# Autodesk Inventor assembly: Overall_Assembly_Rev2
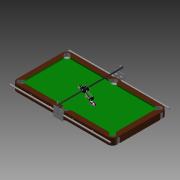
[picture p0: Inventor's stored thumbnail of the model, 180x180]
Saved by Autodesk Inventor 2015 (Build 190159000, 159)
## iProperties
Created: 2016-12-23
Part Number: Overall_Assembly_Rev2
Document SubType Name: Assembly
Designer: Guy
Author: Guy
## Documents named in this file (6)
- C:\Users\Ernest\Documents\Capstone-Project\doc\CAD\LowLevel_Rev2\Overall_Assembly_Rev2.iam
- C:\Users\Ernest\Documents\Capstone-Project\doc\CAD\Pool Table\Table_Model.ipt
- C:\Users\Ernest\Documents\Capstone-Project\doc\CAD\LowLevel_Rev2\X_rail_Assembly_Rev2.iam
- C:\Users\Ernest\Documents\Capstone-Project\doc\CAD\Rails CAD\lan26-160_silder_pan26-3_Rails_Assembly_Rev2.iam
- C:\Users\Ernest\Documents\Capstone-Project\doc\CAD\LowLevel_Rev2\EE_Assembly_Rev2.iam
- C:\Users\Ernest\Documents\Capstone-Project\doc\CAD\LowLevel_Rev2\Pool_Ball_Stripe.ipt
## Components (8 placed, 6 different names)
1. Table_Model:1 — Mate:1, Angle:1, Flush:1, Flush:2, Mate:2, Angle:2, Flush:3, Flush:4, Tangent:1, Tangent:2
2. X_rail_Assembly_Rev2:1 [sub-assembly] — Mate:2, Angle:2, Flush:3, Flush:4, Mate:3, Mate:6
3. X_rail_Assembly_Rev2:2 [sub-assembly] — Mate:1, Angle:1, Flush:1, Flush:2, Mate:3, Mate:4, Mate:5
4. lan26-160_silder_pan26-3_Rails_Assembly_Rev2:1 [sub-assembly] — Mate:4, Mate:5, Mate:6, Mate:7, Mate:8, Mate:9
5. EE_Assembly_Rev2:1 [sub-assembly] — Mate:7, Mate:8, Mate:9, Mate:10
6. Pool_Ball_Stripe:1 — Tangent:1
7. Pool_Ball_Stripe:2 — Tangent:2
8. ShootingMechanism:1 [sub-assembly] — Mate:10
## Relationships (18: Mate 10, Flush 4, Angle 2, Tangent 2)
- Mate:1: Table_Model:1 ↔ X_rail_Assembly_Rev2:2
- Angle:1 (0 deg): Table_Model:1 ↔ X_rail_Assembly_Rev2:2
- Flush:1 (30 mm): Table_Model:1 ↔ X_rail_Assembly_Rev2:2
- Flush:2: Table_Model:1 ↔ X_rail_Assembly_Rev2:2
- Mate:2: Table_Model:1 ↔ X_rail_Assembly_Rev2:1
- Angle:2 (0 deg): Table_Model:1 ↔ X_rail_Assembly_Rev2:1
- Flush:3: Table_Model:1 ↔ X_rail_Assembly_Rev2:1
- Flush:4 (30 mm): Table_Model:1 ↔ X_rail_Assembly_Rev2:1
- Mate:3: X_rail_Assembly_Rev2:1 ↔ X_rail_Assembly_Rev2:2
- Mate:4: X_rail_Assembly_Rev2:2 ↔ lan26-160_silder_pan26-3_Rails_Assembly_Rev2:1
- Mate:5: X_rail_Assembly_Rev2:2 ↔ lan26-160_silder_pan26-3_Rails_Assembly_Rev2:1
- Mate:6: X_rail_Assembly_Rev2:1 ↔ lan26-160_silder_pan26-3_Rails_Assembly_Rev2:1
- Mate:7: lan26-160_silder_pan26-3_Rails_Assembly_Rev2:1 ↔ EE_Assembly_Rev2:1
- Mate:8: lan26-160_silder_pan26-3_Rails_Assembly_Rev2:1 ↔ EE_Assembly_Rev2:1
- Mate:9: lan26-160_silder_pan26-3_Rails_Assembly_Rev2:1 ↔ EE_Assembly_Rev2:1
- Tangent:1: Table_Model:1 ↔ Pool_Ball_Stripe:1
- Tangent:2: Table_Model:1 ↔ Pool_Ball_Stripe:2
- Mate:10: EE_Assembly_Rev2:1 ↔ ShootingMechanism:1
